# Autodesk Inventor assembly: ASY GBK 3310 central wall shield 5
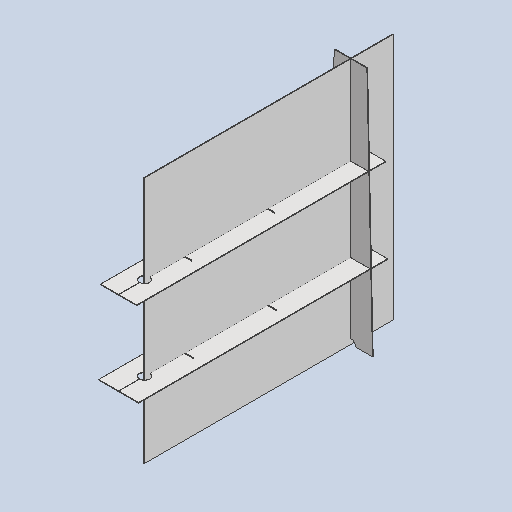
[picture p0: Inventor's stored thumbnail of the model, 512x512]
Saved by Autodesk Inventor 2026 (Build 300175000, 175)
## iProperties
Created: 2026-05-19
Part Number: ASY GBK 3310 central wall shield 5
Document SubType Name: Assembly
Designer: pokla
Mass: 123029 g
Surface Area: 79995.2 cm^2
Volume: 15672.5 cm^3
Density: 7.85 g/cm^3
Author: admin
## Documents named in this file (5)
- C:\Users\pokla\Documents\Inventor\GBK-Gubkinskiy\ASY GBK 3310 central wall shield 5.iam
- C:\Users\pokla\Documents\Inventor\GBK-Gubkinskiy\GBK 3312 stringer 7.ipt
- C:\Users\pokla\Documents\Inventor\GBK-Gubkinskiy\GBK 3315 shield 5.ipt
- C:\Users\pokla\Documents\Inventor\GBK-Gubkinskiy\GBK 3313 stringer 8.ipt
- C:\Users\pokla\Documents\Inventor\GBK-Gubkinskiy\GBK 3311 central third rib.ipt
## Components (7 placed, 4 different names)
1. GBK 3312 stringer 7:1 — Жесткий:1
2. GBK 3315 shield 5:1 — Заподлицо:7, Заподлицо:5, Совмещение:5, Совмещение:2, Заподлицо:1, Совмещение:1, Заподлицо:6, Совмещение:4
3. GBK 3313 stringer 8:1 — Жесткий:2
4. GBK 3312 stringer 7:2 — Жесткий:4
5. GBK 3313 stringer 8:2 — Жесткий:3
6. GBK 3311 central third rib:1 — Заподлицо:6, Заподлицо:4, Совмещение:4, Жесткий:4, Жесткий:3
7. GBK 3311 central third rib:2 — Заподлицо:7, Заподлицо:5, Совмещение:5, Заподлицо:4, Жесткий:1, Жесткий:2
## Relationships (13: Flush 5, Mate 4, WeldJoint 4)
- Заподлицо:7 [Flush]: GBK 3315 shield 5:1 ↔ GBK 3311 central third rib:2
- Заподлицо:5 [Flush] (250 mm): GBK 3315 shield 5:1 ↔ GBK 3311 central third rib:2
- Совмещение:5 [Mate]: GBK 3315 shield 5:1 ↔ GBK 3311 central third rib:2
- Совмещение:2 [Mate]: GBK 3315 shield 5:1
- Заподлицо:1 [Flush]: GBK 3315 shield 5:1
- Совмещение:1 [Mate]: GBK 3315 shield 5:1
- Заподлицо:6 [Flush]: GBK 3315 shield 5:1 ↔ GBK 3311 central third rib:1
- Заподлицо:4 [Flush]: GBK 3311 central third rib:1 ↔ GBK 3311 central third rib:2
- Совмещение:4 [Mate]: GBK 3315 shield 5:1 ↔ GBK 3311 central third rib:1
- Жесткий:1 [WeldJoint] (4 mm): GBK 3312 stringer 7:1 ↔ GBK 3311 central third rib:2
- Жесткий:2 [WeldJoint] (4 mm): GBK 3313 stringer 8:1 ↔ GBK 3311 central third rib:2
- Жесткий:4 [WeldJoint]: GBK 3312 stringer 7:2 ↔ GBK 3311 central third rib:1
- Жесткий:3 [WeldJoint]: GBK 3313 stringer 8:2 ↔ GBK 3311 central third rib:1
